# Autodesk Inventor assembly: gimbal_brushless
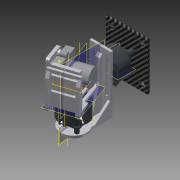
[picture p0: Inventor's stored thumbnail of the model, 180x180]
Saved by Autodesk Inventor 2015 SP1 (Build 190203100, 203)
## iProperties
Created: 2015-08-06
Part Number: gimbal_brushless
Document SubType Name: Assembly
Designer: Alexandre Cherpillod
Mass: 85.7216 g
Surface Area: 256.036 cm^2
Volume: 23.3592 cm^3
Density: 3.66972 g/cm^3
Author: Alexandre Cherpillod
## Documents named in this file (9)
- D:\_windows\_github_doc\MAVRIC\Mechanics\myCopter_CAD\Inventor\Gimbal_Brushless\gimbal_brushless.iam
- D:\_windows\_github_doc\MAVRIC\Mechanics\myCopter_CAD\Inventor\Gimbal_Brushless\carbon_bump_brushless.ipt
- D:\_windows\_github_doc\MAVRIC\Mechanics\myCopter_CAD\Inventor\Gimbal_Brushless\motor_GM1806-80T_skyPro.iam
- D:\_windows\_github_doc\MAVRIC\Mechanics\myCopter_CAD\Inventor\Gimbal_Brushless\gimbal_yaw_brushless.ipt
- D:\_windows\_github_doc\MAVRIC\Mechanics\myCopter_CAD\Inventor\Gimbal_Brushless\gimbal_pitch_brushless.ipt
- D:\_windows\_github_doc\MAVRIC\Mechanics\myCopter_CAD\Inventor\Gimbal_Brushless\camera_support_prz.ipt
- D:\_windows\_github_doc\MAVRIC\Mechanics\myCopter_CAD\Inventor\Gimbal_third_party\camera_prz.ipt
- D:\_windows\_github_doc\MAVRIC\Mechanics\myCopter_CAD\Inventor\Gimbal_Brushless\camera_support_.Fatshark_600TVLipt.ipt
- D:\_windows\_github_doc\MAVRIC\Mechanics\myCopter_CAD\Inventor\Gimbal_third_party\camera_Fatshark_600TVL.ipt
## Components (9 placed, 8 different names)
1. carbon_bump_brushless:1 — Mate:1, Mate:2, Mate:3
2. motor_GM1806-80T_skyPro:1 [sub-assembly] — Mate:1, Mate:2, Mate:3, Flush:1, Mate:4, Flush:4
3. gimbal_yaw_brushless:1 — Flush:1, Mate:4, Mate:5, Mate:6, Mate:7, Flush:4
4. motor_GM1806-80T_skyPro:2 [sub-assembly] — Mate:5, Mate:6, Mate:7, Mate:8, Mate:9, Flush:2
5. gimbal_pitch_brushless:1 — Mate:8, Mate:9, Mate:10, Mate:11, Flush:2, Flush:3, Mate:15, Mate:16, Flush:5
6. camera_support_prz:1 — Mate:10, Mate:11, Mate:12, Mate:13, Mate:14, Flush:3
7. camera_prz:1 — Mate:12, Mate:13, Mate:14
8. camera_support_.Fatshark_600TVLipt:1 — Mate:15, Mate:16, Flush:5, Mate:17, Mate:18, Mate:19
9. camera_Fatshark_600TVL:1 — Mate:17, Mate:18, Mate:19
## Relationships (24: Mate 19, Flush 5)
- Mate:1: carbon_bump_brushless:1 ↔ motor_GM1806-80T_skyPro:1
- Mate:2: carbon_bump_brushless:1 ↔ motor_GM1806-80T_skyPro:1
- Mate:3: carbon_bump_brushless:1 ↔ motor_GM1806-80T_skyPro:1
- Flush:1: motor_GM1806-80T_skyPro:1 ↔ gimbal_yaw_brushless:1
- Mate:4: motor_GM1806-80T_skyPro:1 ↔ gimbal_yaw_brushless:1
- Mate:5: gimbal_yaw_brushless:1 ↔ motor_GM1806-80T_skyPro:2
- Mate:6: gimbal_yaw_brushless:1 ↔ motor_GM1806-80T_skyPro:2
- Mate:7: gimbal_yaw_brushless:1 ↔ motor_GM1806-80T_skyPro:2
- Mate:8: motor_GM1806-80T_skyPro:2 ↔ gimbal_pitch_brushless:1
- Mate:9: motor_GM1806-80T_skyPro:2 ↔ gimbal_pitch_brushless:1
- Mate:10: gimbal_pitch_brushless:1 ↔ camera_support_prz:1
- Mate:11: gimbal_pitch_brushless:1 ↔ camera_support_prz:1
- Mate:12: camera_support_prz:1 ↔ camera_prz:1
- Mate:13: camera_support_prz:1 ↔ camera_prz:1
- Mate:14: camera_support_prz:1 ↔ camera_prz:1
- Flush:2 (-16 mm): motor_GM1806-80T_skyPro:2 ↔ gimbal_pitch_brushless:1
- Flush:3 (-8 mm): gimbal_pitch_brushless:1 ↔ camera_support_prz:1
- Flush:4 (-31 mm): motor_GM1806-80T_skyPro:1 ↔ gimbal_yaw_brushless:1
- Mate:15: gimbal_pitch_brushless:1 ↔ camera_support_.Fatshark_600TVLipt:1
- Mate:16: gimbal_pitch_brushless:1 ↔ camera_support_.Fatshark_600TVLipt:1
- Flush:5 (2 mm): gimbal_pitch_brushless:1 ↔ camera_support_.Fatshark_600TVLipt:1
- Mate:17: camera_support_.Fatshark_600TVLipt:1 ↔ camera_Fatshark_600TVL:1
- Mate:18: camera_support_.Fatshark_600TVLipt:1 ↔ camera_Fatshark_600TVL:1
- Mate:19: camera_support_.Fatshark_600TVLipt:1 ↔ camera_Fatshark_600TVL:1
